# Autodesk Inventor assembly: 소형 커피포트
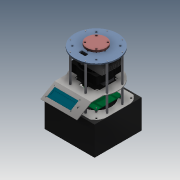
[picture p0: Inventor's stored thumbnail of the model, 180x180]
Saved by Autodesk Inventor 2018 (Build 220112000, 112)
## iProperties
Created: 2018-10-26
Part Number: 소형 커피포트
Material: 일반
Document SubType Name: Assembly
Designer: dhksr
Author: dhksr
## Documents named in this file (14)
- D:\CloudStation\2_프로젝트 백업\소형 커피포트\디자인\소형 커피포트.iam
- D:\CloudStation\2_프로젝트 백업\소형 커피포트\디자인\모터드라이버.ipt
- D:\CloudStation\2_프로젝트 백업\소형 커피포트\디자인\접촉부 철판가공.ipt
- D:\CloudStation\2_프로젝트 백업\소형 커피포트\디자인\펠티어 소자.ipt
- D:\CloudStation\2_프로젝트 백업\소형 커피포트\디자인\CPU쿨러.ipt
- D:\CloudStation\2_프로젝트 백업\소형 커피포트\디자인\CPU면 철판가공 - 복사본.ipt
- D:\CloudStation\2_프로젝트 백업\소형 커피포트\디자인\30mm지지대.ipt
- D:\CloudStation\2_프로젝트 백업\소형 커피포트\디자인\50mm지지대.ipt
- D:\CloudStation\2_프로젝트 백업\소형 커피포트\디자인\모터드라이버 지지대 철판가공.ipt
- D:\CloudStation\2_프로젝트 백업\소형 커피포트\디자인\제어회로 지지대 철판가공.ipt
- D:\CloudStation\2_프로젝트 백업\소형 커피포트\디자인\제어회로.ipt
- D:\CloudStation\2_프로젝트 백업\소형 커피포트\디자인\6mm지지대.ipt
- D:\CloudStation\2_프로젝트 백업\소형 커피포트\디자인\파워서플라이.ipt
- D:\CloudStation\2_프로젝트 백업\소형 커피포트\디자인\1806LCD.ipt
## Components (38 placed, 13 different names)
1. 모터드라이버:1 — 메이트:53, 메이트:54, 메이트:57
2. 펠티어 소자:1 — 메이트:4, 각도:1, 메이트:12, 메이트:13, 플러쉬:1, 메이트:84
3. CPU쿨러:1 — 메이트:3, 각도:1, 메이트:77, 메이트:78
4. CPU면 철판가공 - 복사본:1 — 메이트:3, 메이트:4, 메이트:12, 메이트:13, 메이트:33, 메이트:34, 메이트:35, 메이트:36, 메이트:38, 메이트:39, 메이트:42, 메이트:43, 메이트:44, 메이트:45, 메이트:46, 메이트:47, 메이트:48, 메이트:49, 메이트:50, 메이트:51, 메이트:77, 메이트:78, 메이트:85, 메이트:86
5. 30mm지지대:2
6. 50mm지지대:2 — 메이트:39, 메이트:46
7. 30mm지지대:3
8. 50mm지지대:3 — 메이트:38, 메이트:45
9. 30mm지지대:4
10. 50mm지지대:4 — 메이트:43, 메이트:44
11. 30mm지지대:5 — 메이트:60, 메이트:61
12. 50mm지지대:5 — 메이트:36, 메이트:51
13. 30mm지지대:6
14. 50mm지지대:6 — 메이트:34, 메이트:49
15. 30mm지지대:7
16. 50mm지지대:7 — 메이트:35, 메이트:50
17. 30mm지지대:8
18. 50mm지지대:8 — 메이트:33, 메이트:48
19. 30mm지지대:9 — 메이트:73
20. 50mm지지대:9 — 메이트:42, 메이트:47
21. 모터드라이버 지지대 철판가공:1 — 메이트:53, 메이트:54, 메이트:57, 메이트:60, 메이트:62, 메이트:72, 메이트:73, 메이트:76, 메이트:90, 메이트:91, 메이트:92
22. 제어회로:1 — 메이트:71, 메이트:80, 메이트:81, 메이트:83
23. 제어회로 지지대 철판가공:2 — 메이트:74, 메이트:75, 메이트:76, 메이트:79, 메이트:82, 메이트:83, 메이트:87, 메이트:88, 메이트:89
24. 접촉부 철판가공:2 — 메이트:84, 메이트:85, 메이트:86
25. 파워서플라이:1 — 메이트:87, 메이트:88, 메이트:89
26. 1806LCD:1 — 메이트:90, 메이트:91, 메이트:92
27. 50mm지지대:12 — 메이트:61, 메이트:62, 메이트:72, 메이트:74, 메이트:75
28. 50mm지지대:13
29. 50mm지지대:14
30. 50mm지지대:15
31. 50mm지지대:16
32. 50mm지지대:17
33. 50mm지지대:18
34. 50mm지지대:19
35. 6mm지지대:1 — 메이트:71, 메이트:79, 메이트:80, 메이트:81, 메이트:82
36. 6mm지지대:2
37. 6mm지지대:3
38. 6mm지지대:4
## Component patterns: (8 elements, first: 50mm지지대:12), (4 elements, first: 6mm지지대:1)
## Relationships (74: Mate 64, Flush 9, Angle 1)
- 메이트:3 [Mate]: CPU쿨러:1 ↔ CPU면 철판가공 - 복사본:1
- 메이트:4 [Mate]: 펠티어 소자:1 ↔ CPU면 철판가공 - 복사본:1
- 각도:1 [Angle] (45 deg): 펠티어 소자:1 ↔ CPU쿨러:1
- 메이트:12 [Mate] (-20 mm): 펠티어 소자:1 ↔ CPU면 철판가공 - 복사본:1
- 메이트:13 [Mate] (-20 mm): 펠티어 소자:1 ↔ CPU면 철판가공 - 복사본:1
- 플러쉬:1 [Flush] (-20 mm): 펠티어 소자:1
- [Mate]: 30mm지지대:2 ↔ 50mm지지대:2
- [Mate]: 30mm지지대:2 ↔ 50mm지지대:2
- [Flush]: 30mm지지대:2 ↔ 50mm지지대:2
- [Mate]: 30mm지지대:3 ↔ 50mm지지대:3
- [Mate]: 30mm지지대:3 ↔ 50mm지지대:3
- [Flush]: 30mm지지대:3 ↔ 50mm지지대:3
- [Mate]: 30mm지지대:4 ↔ 50mm지지대:4
- [Mate]: 30mm지지대:4 ↔ 50mm지지대:4
- [Flush]: 30mm지지대:4 ↔ 50mm지지대:4
- [Mate]: 30mm지지대:5 ↔ 50mm지지대:5
- [Mate]: 30mm지지대:5 ↔ 50mm지지대:5
- [Flush]: 30mm지지대:5 ↔ 50mm지지대:5
- [Mate]: 30mm지지대:6 ↔ 50mm지지대:6
- [Mate]: 30mm지지대:6 ↔ 50mm지지대:6
- [Flush]: 30mm지지대:6 ↔ 50mm지지대:6
- [Mate]: 30mm지지대:7 ↔ 50mm지지대:7
- [Mate]: 30mm지지대:7 ↔ 50mm지지대:7
- [Flush]: 30mm지지대:7 ↔ 50mm지지대:7
- [Mate]: 30mm지지대:8 ↔ 50mm지지대:8
- [Mate]: 30mm지지대:8 ↔ 50mm지지대:8
- [Flush]: 30mm지지대:8 ↔ 50mm지지대:8
- 메이트:33 [Mate]: CPU면 철판가공 - 복사본:1 ↔ 50mm지지대:8
- 메이트:34 [Mate]: CPU면 철판가공 - 복사본:1 ↔ 50mm지지대:6
- 메이트:35 [Mate]: CPU면 철판가공 - 복사본:1 ↔ 50mm지지대:7
- 메이트:36 [Mate]: CPU면 철판가공 - 복사본:1 ↔ 50mm지지대:5
- 메이트:38 [Mate]: CPU면 철판가공 - 복사본:1 ↔ 50mm지지대:3
- 메이트:39 [Mate]: CPU면 철판가공 - 복사본:1 ↔ 50mm지지대:2
- [Mate]: 30mm지지대:9 ↔ 50mm지지대:9
- [Mate]: 30mm지지대:9 ↔ 50mm지지대:9
- [Flush]: 30mm지지대:9 ↔ 50mm지지대:9
- 메이트:42 [Mate]: CPU면 철판가공 - 복사본:1 ↔ 50mm지지대:9
- 메이트:43 [Mate]: CPU면 철판가공 - 복사본:1 ↔ 50mm지지대:4
- 메이트:44 [Mate]: CPU면 철판가공 - 복사본:1 ↔ 50mm지지대:4
- 메이트:45 [Mate]: CPU면 철판가공 - 복사본:1 ↔ 50mm지지대:3
- 메이트:46 [Mate]: CPU면 철판가공 - 복사본:1 ↔ 50mm지지대:2
- 메이트:47 [Mate]: CPU면 철판가공 - 복사본:1 ↔ 50mm지지대:9
- 메이트:48 [Mate]: CPU면 철판가공 - 복사본:1 ↔ 50mm지지대:8
- 메이트:49 [Mate]: CPU면 철판가공 - 복사본:1 ↔ 50mm지지대:6
- 메이트:50 [Mate]: CPU면 철판가공 - 복사본:1 ↔ 50mm지지대:7
- 메이트:51 [Mate]: CPU면 철판가공 - 복사본:1 ↔ 50mm지지대:5
- 메이트:53 [Mate]: 모터드라이버:1 ↔ 모터드라이버 지지대 철판가공:1
- 메이트:54 [Mate]: 모터드라이버:1 ↔ 모터드라이버 지지대 철판가공:1
- 메이트:57 [Mate]: 모터드라이버:1 ↔ 모터드라이버 지지대 철판가공:1
- 메이트:60 [Mate]: 30mm지지대:5 ↔ 모터드라이버 지지대 철판가공:1
- 메이트:61 [Mate]: 30mm지지대:5 ↔ 50mm지지대:12
- 메이트:62 [Mate]: 모터드라이버 지지대 철판가공:1 ↔ 50mm지지대:12
- 메이트:71 [Mate]: 제어회로:1 ↔ 6mm지지대:1
- 메이트:72 [Mate]: 모터드라이버 지지대 철판가공:1 ↔ 50mm지지대:12
- 메이트:73 [Mate]: 30mm지지대:9 ↔ 모터드라이버 지지대 철판가공:1
- 메이트:74 [Mate]: 제어회로 지지대 철판가공:2 ↔ 50mm지지대:12
- 메이트:75 [Mate]: 제어회로 지지대 철판가공:2 ↔ 50mm지지대:12
- 메이트:76 [Mate]: 모터드라이버 지지대 철판가공:1 ↔ 제어회로 지지대 철판가공:2
- 메이트:77 [Mate]: CPU쿨러:1 ↔ CPU면 철판가공 - 복사본:1
- 메이트:78 [Mate]: CPU쿨러:1 ↔ CPU면 철판가공 - 복사본:1
- 메이트:79 [Mate]: 제어회로 지지대 철판가공:2 ↔ 6mm지지대:1
- 메이트:80 [Mate]: 제어회로:1 ↔ 6mm지지대:1
- 메이트:81 [Mate]: 제어회로:1 ↔ 6mm지지대:1
- 메이트:82 [Mate]: 제어회로 지지대 철판가공:2 ↔ 6mm지지대:1
- 메이트:83 [Mate]: 제어회로:1 ↔ 제어회로 지지대 철판가공:2
- 메이트:84 [Mate]: 펠티어 소자:1 ↔ 접촉부 철판가공:2
- 메이트:85 [Mate]: CPU면 철판가공 - 복사본:1 ↔ 접촉부 철판가공:2
- 메이트:86 [Mate]: CPU면 철판가공 - 복사본:1 ↔ 접촉부 철판가공:2
- 메이트:87 [Mate]: 제어회로 지지대 철판가공:2 ↔ 파워서플라이:1
- 메이트:88 [Mate]: 제어회로 지지대 철판가공:2 ↔ 파워서플라이:1
- 메이트:89 [Mate]: 제어회로 지지대 철판가공:2 ↔ 파워서플라이:1
- 메이트:90 [Mate] (6 mm): 모터드라이버 지지대 철판가공:1 ↔ 1806LCD:1
- 메이트:91 [Mate]: 모터드라이버 지지대 철판가공:1 ↔ 1806LCD:1
- 메이트:92 [Mate]: 모터드라이버 지지대 철판가공:1 ↔ 1806LCD:1
## Named parameters: d29_d26 = 0 mm, d30_d27 = 0 mm, d31_d28 = 0 mm, d32_d26 = 0 mm, d33_d27 = 0 mm, d34_d28 = 0 mm, d35_d26 = 0 mm, d36_d27 = 0 mm, d37_d28 = 0 mm, d38_d26 = 0 mm, d39_d27 = 0 mm, d40_d28 = 0 mm, d41_d26 = 0 mm, d42_d27 = 0 mm, d43_d28 = 0 mm, d44_d26 = 0 mm, d45_d27 = 0 mm, d46_d28 = 0 mm, d47_d26 = 0 mm, d48_d27 = 0 mm, d49_d28 = 0 mm, d60_d35_d26 = 0 mm, d61_d36_d27 = 0 mm, d62_d37_d28 = 0 mm
